# Autodesk Inventor assembly: BNO055
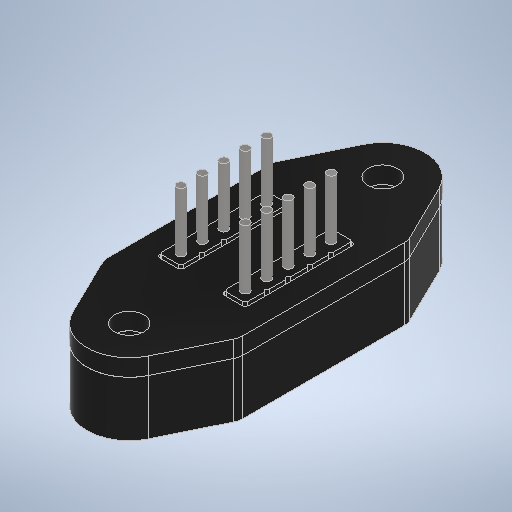
[picture p0: Inventor's stored thumbnail of the model, 512x512]
Saved by Autodesk Inventor 2025.1 (Build 291241020, 241B)
## iProperties
Created: 2024-08-31
Part Number: BNO055
Document SubType Name: Assembly
Designer: 8326d
Author: 8326d
## Documents named in this file (4)
- C:\Users\8326d\Documents\hobby\CAD\General-Purpose-Robot\circuits\BNO055.iam
- C:\Users\8326d\Documents\hobby\CAD\General-Purpose-Robot\circuits\3D_bno055_bottom.ipt
- C:\Users\8326d\Documents\hobby\CAD\General-Purpose-Robot\circuits\3D_bno055_top.ipt
- C:\Users\8326d\Documents\hobby\CAD\General-Purpose-Robot\circuits\bno055_module.ipt
## Components (3 placed, 3 different names)
1. 3D_bno055_bottom:1 — 挿入:1, 挿入:2
2. 3D_bno055_top:1 — メイト:1, メイト:2, メイト:3, 挿入:1, 挿入:2
3. bno055_module:1 — メイト:1, メイト:2, メイト:3
## Relationships (5: Mate 3, Insert 2)
- メイト:1 [Mate]: 3D_bno055_top:1 ↔ bno055_module:1
- メイト:2 [Mate] (0.18 mm): 3D_bno055_top:1 ↔ bno055_module:1
- メイト:3 [Mate] (0.17 mm): 3D_bno055_top:1 ↔ bno055_module:1
- 挿入:1 [Insert]: 3D_bno055_bottom:1 ↔ 3D_bno055_top:1
- 挿入:2 [Insert]: 3D_bno055_bottom:1 ↔ 3D_bno055_top:1
